# Autodesk Inventor assembly: Assembly
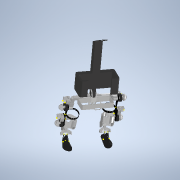
[picture p0: Inventor's stored thumbnail of the model, 180x180]
Saved by Autodesk Inventor 2021 (Build 250183000, 183)
## iProperties
Created: 2021-03-21
Part Number: Assembly
Document SubType Name: Assembly
Designer: 91730
Author: 91730
## Documents named in this file (30)
- D:\Model\Mechanical Leg Exoskeleton\Assembly.iam
- D:\Model\Mohit Rajput\Rotatory Hinge 1.ipt
- D:\Model\Mohit Rajput\Rotatory Hinge 2.ipt
- D:\Model\Mohit Rajput\Rotatory Hinge 3.ipt
- D:\Model\Mukul Raj\Shoes (Lower part).ipt
- D:\Model\Narla Karthikeya\Gear and handle.ipt
- D:\Model\Naval Jaggi\Waist Adjustment Part.ipt
- D:\Model\Nesar Joshi\Hip Belt.ipt
- D:\Model\Nidhi Upasani\Waist Link.ipt
- D:\Model\Nilanshi Patel\Thigh Support.ipt
- D:\Model\Sahil Nayak\TRUNK.ipt
- D:\Model\Naval Jaggi\Waist Adjustment Part_MIR.ipt
- D:\Model\Nilanshi Patel\Thigh Support_MIR.ipt
- D:\Model\Mohit Rajput\Rotatory Hinge 2_MIR.ipt
- D:\Model\Mihika Jadhav\Shoes (upper part)_MIR.ipt
- D:\Model\Mukul Raj\Shoes (Lower part)_MIR.ipt
- D:\Model\Mohit Rajput\Rotatory Hinge 1_MIR.ipt
- D:\Model\Mohit Rajput\Rotatory Hinge 3_MIR.ipt
- D:\Model\Narla Karthikeya\Gear and handle_MIR.ipt
- D:\Model\Mohit Rajput\Rotatory Hinge 1_CPY.ipt
- D:\Model\Mohit Rajput\Rotatory Hinge 3_CPY.ipt
- D:\Model\Narla Karthikeya\Gear and handle_CPY.ipt
- D:\Model\Mohit Rajput\Rotatory Hinge 1_MIR_CPY.ipt
- D:\Model\Mohit Rajput\Rotatory Hinge 3_MIR_CPY.ipt
- D:\Model\Narla Karthikeya\Gear and handle_MIR_CPY.ipt
- D:\Model\Mechanical Leg Exoskeleton\Rotatory Hinge 4-01.ipt
- D:\Model\Mohit Rajput\Rotatory Hinge 4.ipt
- D:\Model\Mumuksh Tayal\CRUS FRAME.ipt
- D:\Model\Mumuksh Tayal\CRUS FRAME_MIR.ipt
- D:\Model\Mihika Jadhav\Shoes (upper part)_MIR_MIR.ipt
## Components (31 placed, 27 different names)
1. Rotatory Hinge 1:1 — Mate:54, Mate:55
2. Rotatory Hinge 2:1 — Mate:6, Flush:5, Mate:20, Mate:22, Mate:23
3. Spur Gear1:1 — Mate:40, Mate:41
4. Gear and handle:1 — Mate:40, Mate:41, Mate:44, Flush:11, Mate:45
5. Waist Adjustment Part:1 — Mate:3, Mate:4, Mate:5, Flush:2, Mate:6, Mate:7, Mate:13, Flush:5, Mate:60, Flush:12, Mate:61
6. Hip Belt:1 — Mate:10, Flush:3, Flush:4
7. Waist Link:1 — Mate:1, Mate:2, Flush:1, Mate:3, Flush:2, Mate:10, Flush:3, Flush:4
8. Thigh Support:1 — Mate:7, Mate:13, Flush:9, Mate:19, Flush:10, Mate:21, Mate:28, Mate:46, Mate:47
9. TRUNK:1 — Mate:1, Mate:2, Flush:1
10. Waist Adjustment Part_MIR:1 — Mate:4, Mate:5, Mate:8, Mate:14, Flush:6, Mate:44, Flush:11, Mate:45
11. Thigh Support_MIR:1 — Mate:9, Mate:14, Mate:18, Flush:7, Flush:8, Mate:25, Mate:32, Mate:51, Mate:52
12. Rotatory Hinge 2_MIR:1 — Mate:8, Mate:9, Flush:6, Mate:24, Mate:26, Mate:27
13. Rotatory Hinge 1_MIR:1 — Mate:26, Mate:27
14. Rotatory Hinge 3_MIR:1 — Mate:42, Mate:43
15. Gear and handle_MIR:1 — Mate:42, Mate:43, Mate:60, Flush:12, Mate:61
16. Rotatory Hinge 1_CPY:1 — Mate:22, Mate:23
17. Spur Gear1:2 — Mate:36, Mate:37
18. Gear and handle_CPY:1 — Mate:18, Flush:7, Flush:8, Mate:36, Mate:37
19. Rotatory Hinge 1_MIR_CPY:1 — Mate:49, Mate:50
20. Rotatory Hinge 3_MIR_CPY:1 — Mate:38, Mate:39
21. Gear and handle_MIR_CPY:1 — Flush:9, Mate:19, Flush:10, Mate:38, Mate:39
22. Spur Gear2:1 — Mate:24, Mate:25
23. Spur Gear2:2 — Mate:20, Mate:21
24. Spur Gear2:3 — Mate:28, Mate:48
25. Spur Gear2:4 — Mate:32, Mate:53
26. Shoes (upper part)_MIR:1 — Mate:56, Mate:58
27. CRUS FRAME:1 — Mate:51, Mate:52, Mate:53, Mate:54, Mate:55, Mate:57, Flush:14
28. CRUS FRAME_MIR:1 — Mate:46, Mate:47, Mate:48, Mate:49, Mate:50, Mate:56, Flush:13
29. Shoes (upper part)_MIR_MIR:1 — Mate:57, Mate:59
30. Shoes (Lower part):1 — Mate:59, Flush:14
31. Shoes (Lower part)_MIR:1 — Mate:58, Flush:13
## Relationships (64: Mate 50, Flush 14)
- Mate:1: Waist Link:1 ↔ TRUNK:1
- Mate:2: Waist Link:1 ↔ TRUNK:1
- Flush:1: Waist Link:1 ↔ TRUNK:1
- Mate:3: Waist Adjustment Part:1 ↔ Waist Link:1
- Mate:4: Waist Adjustment Part:1 ↔ Waist Adjustment Part_MIR:1
- Mate:5: Waist Adjustment Part:1 ↔ Waist Adjustment Part_MIR:1
- Flush:2 (80 mm): Waist Adjustment Part:1 ↔ Waist Link:1
- Mate:6: Rotatory Hinge 2:1 ↔ Waist Adjustment Part:1
- Mate:7: Waist Adjustment Part:1 ↔ Thigh Support:1
- Mate:8: Waist Adjustment Part_MIR:1 ↔ Rotatory Hinge 2_MIR:1
- Mate:9: Thigh Support_MIR:1 ↔ Rotatory Hinge 2_MIR:1
- Mate:10: Hip Belt:1 ↔ Waist Link:1
- Flush:3: Hip Belt:1 ↔ Waist Link:1
- Flush:4: Hip Belt:1 ↔ Waist Link:1
- Mate:13: Waist Adjustment Part:1 ↔ Thigh Support:1
- Mate:14: Waist Adjustment Part_MIR:1 ↔ Thigh Support_MIR:1
- Flush:5: Rotatory Hinge 2:1 ↔ Waist Adjustment Part:1
- Flush:6: Waist Adjustment Part_MIR:1 ↔ Rotatory Hinge 2_MIR:1
- Mate:18: Thigh Support_MIR:1 ↔ Gear and handle_CPY:1
- Flush:7: Thigh Support_MIR:1 ↔ Gear and handle_CPY:1
- Flush:8: Thigh Support_MIR:1 ↔ Gear and handle_CPY:1
- Flush:9: Thigh Support:1 ↔ Gear and handle_MIR_CPY:1
- Mate:19: Thigh Support:1 ↔ Gear and handle_MIR_CPY:1
- Flush:10: Thigh Support:1 ↔ Gear and handle_MIR_CPY:1
- Mate:20: Rotatory Hinge 2:1 ↔ Spur Gear2:2
- Mate:21: Thigh Support:1 ↔ Spur Gear2:2
- Mate:22: Rotatory Hinge 2:1 ↔ Rotatory Hinge 1_CPY:1
- Mate:23: Rotatory Hinge 2:1 ↔ Rotatory Hinge 1_CPY:1
- Mate:24: Rotatory Hinge 2_MIR:1 ↔ Spur Gear2:1
- Mate:25: Thigh Support_MIR:1 ↔ Spur Gear2:1
- Mate:26: Rotatory Hinge 2_MIR:1 ↔ Rotatory Hinge 1_MIR:1
- Mate:27: Rotatory Hinge 2_MIR:1 ↔ Rotatory Hinge 1_MIR:1
- Mate:28: Thigh Support:1 ↔ Spur Gear2:3
- Mate:32: Thigh Support_MIR:1 ↔ Spur Gear2:4
- Mate:36: Spur Gear1:2 ↔ Gear and handle_CPY:1
- Mate:37: Spur Gear1:2 ↔ Gear and handle_CPY:1
- Mate:38: Rotatory Hinge 3_MIR_CPY:1 ↔ Gear and handle_MIR_CPY:1
- Mate:39: Rotatory Hinge 3_MIR_CPY:1 ↔ Gear and handle_MIR_CPY:1
- Mate:40: Spur Gear1:1 ↔ Gear and handle:1
- Mate:41: Spur Gear1:1 ↔ Gear and handle:1
- Mate:42: Rotatory Hinge 3_MIR:1 ↔ Gear and handle_MIR:1
- Mate:43: Rotatory Hinge 3_MIR:1 ↔ Gear and handle_MIR:1
- Mate:44: Gear and handle:1 ↔ Waist Adjustment Part_MIR:1
- Flush:11: Gear and handle:1 ↔ Waist Adjustment Part_MIR:1
- Mate:45 (-10 mm): Gear and handle:1 ↔ Waist Adjustment Part_MIR:1
- Mate:46: Thigh Support:1 ↔ CRUS FRAME_MIR:1
- Mate:47: Thigh Support:1 ↔ CRUS FRAME_MIR:1
- Mate:48: Spur Gear2:3 ↔ CRUS FRAME_MIR:1
- Mate:49: Rotatory Hinge 1_MIR_CPY:1 ↔ CRUS FRAME_MIR:1
- Mate:50: Rotatory Hinge 1_MIR_CPY:1 ↔ CRUS FRAME_MIR:1
- Mate:51: Thigh Support_MIR:1 ↔ CRUS FRAME:1
- Mate:52: Thigh Support_MIR:1 ↔ CRUS FRAME:1
- Mate:53: Spur Gear2:4 ↔ CRUS FRAME:1
- Mate:54: Rotatory Hinge 1:1 ↔ CRUS FRAME:1
- Mate:55: Rotatory Hinge 1:1 ↔ CRUS FRAME:1
- Mate:56: Shoes (upper part)_MIR:1 ↔ CRUS FRAME_MIR:1
- Mate:57: CRUS FRAME:1 ↔ Shoes (upper part)_MIR_MIR:1
- Mate:58: Shoes (upper part)_MIR:1 ↔ Shoes (Lower part)_MIR:1
- Mate:59: Shoes (upper part)_MIR_MIR:1 ↔ Shoes (Lower part):1
- Mate:60: Waist Adjustment Part:1 ↔ Gear and handle_MIR:1
- Flush:12: Waist Adjustment Part:1 ↔ Gear and handle_MIR:1
- Mate:61 (-10 mm): Waist Adjustment Part:1 ↔ Gear and handle_MIR:1
- Flush:13 (40 mm): CRUS FRAME_MIR:1 ↔ Shoes (Lower part)_MIR:1
- Flush:14 (40 mm): CRUS FRAME:1 ↔ Shoes (Lower part):1
